# Autodesk Inventor assembly: __VK_Stopper_Einheit
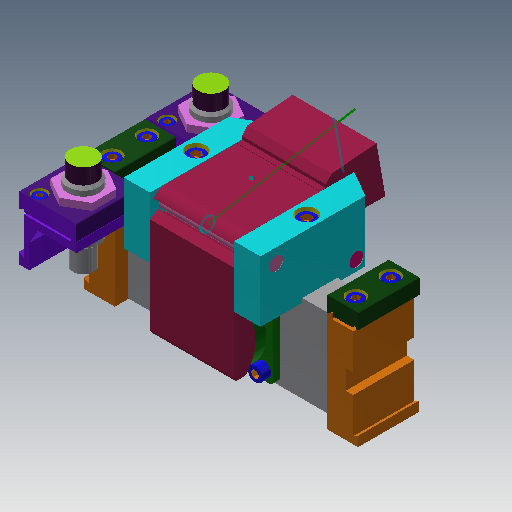
[picture p0: Inventor's stored thumbnail of the model, 512x512]
Saved by Autodesk Inventor 2025.1 (Build 291241000, 241)
## iProperties
Created: 2023-11-18
Part Number: __VK_Stopper_Einheit
Material: Generisch
Document SubType Name: Assembly
Designer: RP
Author: RP
## Documents named in this file (3)
- C:\Users\Erik\Erik\Hochschule\3. Semester\CAD\CAD-Paspa\Useless Box\_Verkettung\__VK_Stopper_Einheit.iam
- C:\Users\Erik\Erik\Hochschule\3. Semester\CAD\CAD-Paspa\Useless Box\_Verkettung\__VK_Stopper.iam
- C:\Users\Erik\Erik\Hochschule\3. Semester\CAD\CAD-Paspa\Useless Box\_Verkettung\__VK_Sensor_Palette_1_0.ipt
## Components (3 placed, 2 different names)
1. __VK_Stopper:1 [sub-assembly] — Fluchtend:1, Fluchtend:2, Fluchtend:3, Fluchtend:4, Fluchtend:5, Fluchtend:6, Passend:1, Passend:2
2. __VK_Sensor_Palette_1_0:1 — Fluchtend:4, Fluchtend:5, Fluchtend:7, Passend:2
3. __VK_Sensor_Palette_1_0:2 — Fluchtend:6, Fluchtend:7, Passend:1
## Relationships (9: Flush 7, Mate 2)
- Fluchtend:1 [Flush]: __VK_Stopper:1
- Fluchtend:2 [Flush]: __VK_Stopper:1
- Fluchtend:3 [Flush]: __VK_Stopper:1
- Fluchtend:4 [Flush]: __VK_Stopper:1 ↔ __VK_Sensor_Palette_1_0:1
- Fluchtend:5 [Flush]: __VK_Stopper:1 ↔ __VK_Sensor_Palette_1_0:1
- Fluchtend:6 [Flush]: __VK_Stopper:1 ↔ __VK_Sensor_Palette_1_0:2
- Fluchtend:7 [Flush]: __VK_Sensor_Palette_1_0:1 ↔ __VK_Sensor_Palette_1_0:2
- Passend:1 [Mate] (1 mm): __VK_Stopper:1 ↔ __VK_Sensor_Palette_1_0:2
- Passend:2 [Mate] (1 mm): __VK_Stopper:1 ↔ __VK_Sensor_Palette_1_0:1
